# Autodesk Inventor assembly: tanks
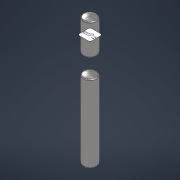
[picture p0: Inventor's stored thumbnail of the model, 180x180]
Saved by Autodesk Inventor 2021 (Build 250183000, 183)
## iProperties
Created: 2020-12-02
Part Number: tanks
Document SubType Name: Assembly
Designer: henry
Author: henry
## Documents named in this file (10)
- C:\Users\henry\Desktop\rocket\cad\tanks.iam
- C:\Users\henry\Desktop\rocket\cad\fuel tank wall.ipt
- C:\Users\henry\Desktop\rocket\cad\oxidiser tank wall.ipt
- C:\Users\henry\Desktop\rocket\cad\tank endcap.ipt
- C:\Users\henry\Desktop\rocket\cad\tanks\AIP\FEA\dfxzbn38g.fins
- C:\Users\henry\Desktop\rocket\cad\tanks\AIP\FEA\dfxzbn39c.fsat
- C:\Users\henry\Desktop\rocket\cad\tanks\AIP\FEA\dfxzbn39c.ftes
- C:\Users\henry\Desktop\rocket\cad\tanks\AIP\FEA\dfxzbn39c.fwiz
- C:\Users\henry\Desktop\rocket\cad\tanks\AIP\FEA\dfxzbn3a8.fmsh
- C:\Users\henry\Desktop\rocket\cad\tanks\AIP\FEA\dfxzbn3a9.fres
## Components (6 placed, 6 different names)
1. fuel tank wall:1 — Mate:2, Mate:3
2. oxidiser tank wall:1 — Mate:1
3. oxidiser tank lower endcap
4. oxidiser tank upper endcap — Mate:1
5. fuel tank lower endcap — Mate:2
6. fuel tank upper endcap — Mate:3
## Relationships (3: Mate 3)
- Mate:1: oxidiser tank wall:1 ↔ oxidiser tank upper endcap
- Mate:2: fuel tank wall:1 ↔ fuel tank lower endcap
- Mate:3: fuel tank wall:1 ↔ fuel tank upper endcap
## Named parameters: sa_0 = 70000
note: some values were not read from the file. Shown as the stored number, unit unknown: "sa_0".
